# Autodesk Inventor assembly: Сборка ручка
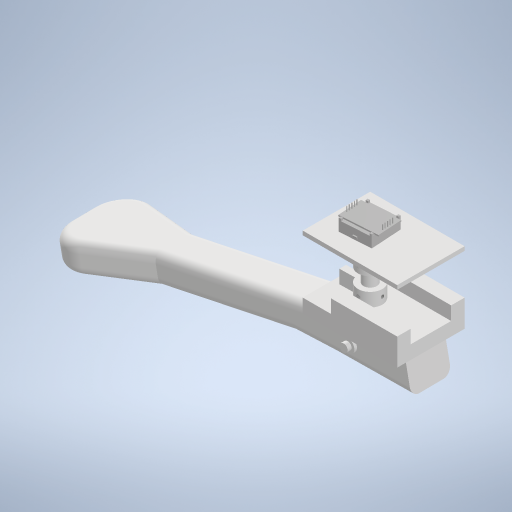
[picture p0: Inventor's stored thumbnail of the model, 512x512]
Saved by Autodesk Inventor 2023 (Build 270158000, 158)
## iProperties
Created: 2022-05-02
Part Number: Сборка ручка
Document SubType Name: Assembly
Designer: User
Author: User
## Documents named in this file (12)
- C:\Users\avkap\Desktop\Стойка\Механизм ручки\Сборка ручка.iam
- C:\Users\avkap\Desktop\Стойка\Механизм ручки\EAW.ipt
- C:\Users\avkap\Desktop\Стойка\Механизм ручки\Вал ручки.ipt
- C:\Users\avkap\Desktop\Стойка\Механизм ручки\Втулка энкодер.ipt
- C:\Users\avkap\Desktop\Стойка\Механизм ручки\Ручка.ipt
- C:\Users\avkap\Desktop\Стойка\Механизм ручки\Стенка.ipt
- C:\Users\avkap\Desktop\Стойка\Механизм ручки\Стопор.ipt
- C:\Users\avkap\Desktop\Стойка\Механизм ручки\Стенка энкодер.ipt
- C:\Users\avkap\Desktop\Стойка\Механизм ручки\Диск.ipt
- C:\Users\avkap\Desktop\Стойка\Механизм ручки\М3х8.ipt
- C:\Users\avkap\Desktop\Стойка\Механизм ручки\Шпилька.ipt
- C:\Users\avkap\Desktop\Стойка\Механизм ручки\Диск конец вала.ipt
## Components (14 placed, 11 different names)
1. EAW:1 — Цилиндрический:4, Совмещение:15
2. Вал ручки:1 — Цилиндрический:12, Цилиндрический:13, Совмещение:13, Цилиндрический:14, Совмещение:17
3. Втулка энкодер:1 — Цилиндрический:3, Цилиндрический:4, Совмещение:16, Совмещение:17
4. Ручка:1 — Совмещение:4, Совмещение:5, Цилиндрический:12, Совмещение:11, Совмещение:12
5. Стенка:1 — Заподлицо:1, Заподлицо:2, Совмещение:4, Цилиндрический:14, Совмещение:14
6. Стопор:1 — Цилиндрический:13, Совмещение:13, Совмещение:14
7. Стенка энкодер:1 — Заподлицо:1, Цилиндрический:3, Заподлицо:2, Совмещение:15, Совмещение:16
8. М3х8:1 — Цилиндрический:11, Совмещение:6
9. Диск:2 — Цилиндрический:10, Совмещение:7, Совмещение:8
10. М3х8:2 — Цилиндрический:9, Цилиндрический:10, Совмещение:7
11. Диск:3 — Цилиндрический:8, Совмещение:9, Совмещение:10, Совмещение:11
12. М3х8:3 — Цилиндрический:7, Цилиндрический:8, Совмещение:10, Совмещение:12
13. Шпилька:1 — Цилиндрический:7, Цилиндрический:9, Совмещение:8, Совмещение:9
14. Диск конец вала:1 — Цилиндрический:11, Совмещение:5, Совмещение:6
## Relationships (26: Mate 14, CylindricalJoint 10, Flush 2)
- Заподлицо:1 [Flush]: Стенка:1 ↔ Стенка энкодер:1
- Цилиндрический:3 [CylindricalJoint]: Втулка энкодер:1 ↔ Стенка энкодер:1
- Цилиндрический:4 [CylindricalJoint]: EAW:1 ↔ Втулка энкодер:1
- Заподлицо:2 [Flush]: Стенка:1 ↔ Стенка энкодер:1
- Цилиндрический:7 [CylindricalJoint]: М3х8:3 ↔ Шпилька:1
- Цилиндрический:8 [CylindricalJoint]: Диск:3 ↔ М3х8:3
- Цилиндрический:9 [CylindricalJoint]: М3х8:2 ↔ Шпилька:1
- Цилиндрический:10 [CylindricalJoint]: Диск:2 ↔ М3х8:2
- Цилиндрический:11 [CylindricalJoint]: М3х8:1 ↔ Диск конец вала:1
- Совмещение:4 [Mate]: Ручка:1 ↔ Стенка:1
- Совмещение:5 [Mate]: Ручка:1 ↔ Диск конец вала:1
- Совмещение:6 [Mate]: М3х8:1 ↔ Диск конец вала:1
- Цилиндрический:12 [CylindricalJoint]: Вал ручки:1 ↔ Ручка:1
- Совмещение:7 [Mate]: Диск:2 ↔ М3х8:2
- Совмещение:8 [Mate]: Диск:2 ↔ Шпилька:1
- Совмещение:9 [Mate]: Диск:3 ↔ Шпилька:1
- Совмещение:10 [Mate]: Диск:3 ↔ М3х8:3
- Совмещение:11 [Mate]: Ручка:1 ↔ Диск:3
- Совмещение:12 [Mate]: Ручка:1 ↔ М3х8:3
- Цилиндрический:13 [CylindricalJoint]: Вал ручки:1 ↔ Стопор:1
- Совмещение:13 [Mate]: Вал ручки:1 ↔ Стопор:1
- Цилиндрический:14 [CylindricalJoint]: Вал ручки:1 ↔ Стенка:1
- Совмещение:14 [Mate]: Стенка:1 ↔ Стопор:1
- Совмещение:15 [Mate]: EAW:1 ↔ Стенка энкодер:1
- Совмещение:16 [Mate]: Втулка энкодер:1 ↔ Стенка энкодер:1
- Совмещение:17 [Mate]: Вал ручки:1 ↔ Втулка энкодер:1
